# Autodesk Inventor assembly: suspensionsystem1
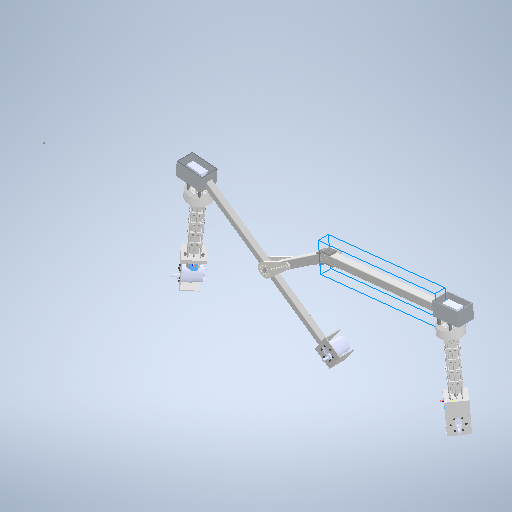
[picture p0: Inventor's stored thumbnail of the model, 512x512]
Saved by Autodesk Inventor 2025.4 (Build 294407000, 407)
## iProperties
Created: 2026-03-25
Part Number: suspensionsystem1
Document SubType Name: Assembly
Designer: hp
Author: hp
## Documents named in this file (51)
- C:\Users\hp\OneDrive\Desktop\Probitymechanicaldocs\suspensionsystem1.iam
- C:\Users\hp\OneDrive\Desktop\Probitymechanicaldocs\suspensionarms.ipt
- C:\Users\hp\OneDrive\Desktop\Probitymechanicaldocs\suspensionaxlebearing.ipt
- C:\Users\hp\OneDrive\Desktop\Probitymechanicaldocs\Controlarm.ipt
- C:\Users\hp\OneDrive\Desktop\Probitymechanicaldocs\rockershaft.ipt
- C:\Users\hp\OneDrive\Desktop\Probitymechanicaldocs\rockerwasher.ipt
- C:\Users\hp\OneDrive\Desktop\Probitymechanicaldocs\suspension2chassisarm.ipt
- C:\Users\hp\OneDrive\Desktop\Probitymechanicaldocs\150degreebracket.ipt
- C:\Users\hp\OneDrive\Desktop\Probitymechanicaldocs\rockerpivotarm.ipt
- C:\Users\hp\OneDrive\Desktop\Probitymechanicaldocs\finalturnmotorcasing.ipt
- C:\Users\hp\OneDrive\Desktop\Probitymechanicaldocs\finalturnmotorservo.ipt
- C:\Users\hp\OneDrive\Desktop\Probitymechanicaldocs\hexcoupling.ipt
- C:\Users\hp\OneDrive\Desktop\Probitymechanicaldocs\couplingload.ipt
- C:\Users\hp\OneDrive\Desktop\Probitymechanicaldocs\sleeve.ipt
- C:\Users\hp\OneDrive\Desktop\Probitymechanicaldocs\verticalaxle.ipt
- C:\Users\hp\OneDrive\Desktop\Probitymechanicaldocs\leadscrew.ipt
- C:\Users\hp\OneDrive\Desktop\Probitymechanicaldocs\leadscrewaxle.ipt
- C:\Users\hp\OneDrive\Desktop\Probitymechanicaldocs\RISE&Fallmotor.ipt
- C:\Users\hp\OneDrive\Desktop\Probitymechanicaldocs\spokes.ipt
- C:\Users\hp\OneDrive\Desktop\Probitymechanicaldocs\liftmotorfloor.ipt
- C:\Users\hp\OneDrive\Desktop\Probitymechanicaldocs\placeholderjoint.ipt
- C:\Users\hp\OneDrive\Desktop\Probitymechanicaldocs\impromptugraphitering.ipt
- C:\Users\hp\OneDrive\Desktop\Probitymechanicaldocs\Placeholderjointouterring.ipt
- C:\Users\hp\OneDrive\Desktop\Probitymechanicaldocs\drivemotorcasing.ipt
- C:\Users\hp\OneDrive\Desktop\Probitymechanicaldocs\extendeddrivemotorcasing.ipt
- C:\Users\hp\OneDrive\Desktop\Probitymechanicaldocs\finaldrivemotor.ipt
- C:\Users\hp\OneDrive\Desktop\Probitymechanicaldocs\150degreesidebracker.ipt
- C:\Users\hp\OneDrive\Documents\Inventor\Content Center Files\R2025\en-US\ISO 4762(2)\ISO 4762 - M4 x 6ISO.ipt
- C:\Users\hp\OneDrive\Documents\Inventor\Content Center Files\R2025\en-US\ISO 7045  H\ISO 7045 - M2.5 x 3_ - 4.8 - H - ISO.ipt
- C:\Users\hp\OneDrive\Documents\Inventor\Content Center Files\R2025\en-US\ISO 1580\ISO 1580 - M2 x 2.5_.ipt
- C:\Users\hp\OneDrive\Desktop\Probitymechanicaldocs\unusedparts\intermediatepin.ipt
- C:\Users\hp\OneDrive\Documents\Inventor\Content Center Files\R2025\en-US\ISO 4035(2)\ISO 4035 - M6 - ISO.ipt
- C:\Users\hp\OneDrive\Desktop\Probitymechanicaldocs\finalturnmotorcasing_MIR.ipt
- C:\Users\hp\OneDrive\Desktop\Probitymechanicaldocs\finalturnmotorservo_MIR.ipt
- C:\Users\hp\OneDrive\Desktop\Probitymechanicaldocs\hexcoupling_MIR.ipt
- C:\Users\hp\OneDrive\Desktop\Probitymechanicaldocs\couplingload_MIR.ipt
- C:\Users\hp\OneDrive\Desktop\Probitymechanicaldocs\sleeve_MIR.ipt
- C:\Users\hp\OneDrive\Desktop\Probitymechanicaldocs\verticalaxle_MIR.ipt
- C:\Users\hp\OneDrive\Desktop\Probitymechanicaldocs\leadscrew_MIR.ipt
- C:\Users\hp\OneDrive\Desktop\Probitymechanicaldocs\leadscrewaxle_MIR.ipt
- C:\Users\hp\OneDrive\Desktop\Probitymechanicaldocs\RISE&Fallmotor_MIR.ipt
- C:\Users\hp\OneDrive\Desktop\Probitymechanicaldocs\spokes_MIR.ipt
- C:\Users\hp\OneDrive\Desktop\Probitymechanicaldocs\liftmotorfloor_MIR.ipt
- C:\Users\hp\OneDrive\Desktop\Probitymechanicaldocs\placeholderjoint_MIR.ipt
- C:\Users\hp\OneDrive\Desktop\Probitymechanicaldocs\impromptugraphitering_MIR.ipt
- C:\Users\hp\OneDrive\Desktop\Probitymechanicaldocs\Placeholderjointouterring_MIR.ipt
- C:\Users\hp\OneDrive\Desktop\Probitymechanicaldocs\extendeddrivemotorcasing_MIR.ipt
- C:\Users\hp\OneDrive\Desktop\Probitymechanicaldocs\finaldrivemotor_MIR.ipt
- C:\Users\hp\OneDrive\Desktop\Probitymechanicaldocs\unusedparts\intermediatepin_MIR.ipt
- C:\Users\hp\OneDrive\Desktop\Probitymechanicaldocs\suspension2chassiscylindricalshaft.ipt
- C:\Users\hp\OneDrive\Desktop\Probitymechanicaldocs\suspension2chassiscylindricalpins.ipt
## Components (217 placed, 50 different names)
1. suspensionarms:1 — Rigid:8, Rotational:130, Rigid:41
2. suspensionaxlebearing:1 — Rotational:3
3. suspensionaxlebearing:2 — Cylindrical:1, Rotational:4, Rotational:130
4. Controlarm:1 — Rotational:9, Rotational:11, Rotational:131
5. Controlarm:2 — Cylindrical:11, Rotational:12, Rotational:132
6. rockershaft:1 — Cylindrical:1
7. rockerwasher:1 — Rotational:4, Rotational:6
8. rockerwasher:2 — Rotational:3, Rotational:5
9. suspensionaxlebearing:3 — Rotational:6, Rotational:11
10. suspensionaxlebearing:4 — Rotational:5, Cylindrical:11
11. suspension2chassisarm:1 — Rotational:9, Rotational:12, Rotational:72, Rotational:131, Rotational:132
12. 150degreebracket:1 — Rigid:16, Rotational:72, Rigid:33
13. rockerpivotarm:1 — Rigid:1, Rigid:16, Rotational:159
14. finalturnmotorcasing:1 — Rigid:1, Rigid:2, Mate:8, Insert:57, Mate:10, Mate:12, Mate:14, Mate:15, Mate:16, Mate:18, Mate:20
15. finalturnmotorservo:1 — Rigid:2, Rotational:13
16. hexcoupling:1 — Rotational:13, Rigid:3
17. couplingload:1 — Rigid:3, Rigid:4
18. sleeve:1 — Rotational:14, Rotational:15, Insert:113, Insert:114, Insert:123, Insert:124, Insert:133, Insert:134, Insert:151, Insert:152
19. verticalaxle:1 — Rigid:4, Rotational:14, Rotational:15, Rotational:16, Cylindrical:12, Rotational:17, Cylindrical:13, Rotational:18, Cylindrical:14, Rotational:19, Rigid:6, Rotational:29, Rotational:30, Rotational:31, Insert:153, Insert:154, Insert:155, Insert:156
20. leadscrew:1 — Rigid:6, Cylindrical:15
21. leadscrewaxle:1 — Rigid:5, Cylindrical:15
22. RISE&Fallmotor:1 — Rigid:5, Rotational:32, Rotational:33
23. sleeve:2 — Rotational:18, Cylindrical:14, Insert:119, Insert:120, Insert:129, Insert:130, Insert:139, Insert:140, Insert:145, Insert:146
24. sleeve:3 — Rotational:19, Rotational:29, Insert:115, Insert:116, Insert:125, Insert:126, Insert:135, Insert:136, Insert:149, Insert:150
25. sleeve:4 — Rotational:17, Cylindrical:13, Insert:121, Insert:122, Insert:131, Insert:132, Insert:141, Insert:142, Insert:143, Insert:144
26. sleeve:5 — Rotational:16, Cylindrical:12, Rigid:7
27. sleeve:6 — Rotational:30, Rotational:31, Insert:117, Insert:118, Insert:127, Insert:128, Insert:137, Insert:138, Insert:147, Insert:148
28. spokes:1 — Rotational:24
29. spokes:2 — Rotational:25
30. spokes:3 — Rotational:23
31. spokes:4 — Rotational:26
32. spokes:5 — Rotational:22
33. spokes:6 — Rotational:28
34. spokes:7 — Rotational:21
35. spokes:8 — Rotational:27
36. liftmotorfloor:1 — Rotational:21, Rotational:22, Rotational:23, Rotational:24, Rotational:25, Rotational:26, Rotational:27, Rotational:28, Rotational:32, Rotational:33, Rotational:62, Mate:5
37. placeholderjoint:1 — Rigid:7, Rotational:34
38. impromptugraphitering:1 — Rotational:34, Rotational:35, Rotational:102
39. Placeholderjointouterring:1 — Rotational:102, Insert:49, Insert:50, Insert:51, Insert:52
40. Placeholderjointouterring:2 — Rotational:35
41. drivemotorcasing:1 — Rigid:8, Rotational:63, Rotational:64, Insert:11, Insert:12, Insert:13, Insert:14, Insert:15, Insert:16
42. extendeddrivemotorcasing:1 — Rotational:62, Mate:5, Rotational:65, Rotational:66, Insert:17, Insert:18, Insert:19, Insert:20, Insert:21, Insert:22
43. finaldrivemotor:1 — Rotational:65, Rotational:66
44. finaldrivemotor:2 — Rotational:63, Rotational:64
45. 150degreesidebracker:1 — Rigid:33, Rigid:43
46. ISO 4762 M4 x 6:1
47. ISO 4762 M4 x 6:2
48. ISO 7045 H M2.5 x 3 - 4.8 - H:7 — Insert:11
49. ISO 7045 H M2.5 x 3 - 4.8 - H:8 — Insert:12
50. ISO 7045 H M2.5 x 3 - 4.8 - H:9 — Insert:13
51. ISO 7045 H M2.5 x 3 - 4.8 - H:10 — Insert:14
52. ISO 7045 H M2.5 x 3 - 4.8 - H:11 — Insert:15
53. ISO 7045 H M2.5 x 3 - 4.8 - H:12 — Insert:16
54. ISO 7045 H M2.5 x 3 - 4.8 - H:13 — Insert:17
55. ISO 7045 H M2.5 x 3 - 4.8 - H:14 — Insert:18
56. ISO 7045 H M2.5 x 3 - 4.8 - H:15 — Insert:19
57. ISO 7045 H M2.5 x 3 - 4.8 - H:16 — Insert:20
58. ISO 7045 H M2.5 x 3 - 4.8 - H:17 — Insert:21
59. ISO 7045 H M2.5 x 3 - 4.8 - H:18 — Insert:22
60. ISO 1580 M2 x 2.5:3
61. ISO 1580 M2 x 2.5:4
62. ISO 1580 M2 x 2.5:5
63. ISO 1580 M2 x 2.5:26
64. intermediatepin:1 — Insert:49, Mate:11, Mate:13
65. intermediatepin:2 — Insert:50, Mate:9
66. intermediatepin:3 — Insert:52, Mate:7, Mate:19
67. intermediatepin:5 — Insert:51, Mate:17
68. ISO 4035 M6:1 — Mate:7, Mate:8
69. ISO 4035 M6:2 — Insert:57
70. ISO 4035 M6:3 — Mate:9, Mate:10
71. ISO 4035 M6:4 — Mate:11, Mate:12
72. ISO 4035 M6:5 — Mate:13, Mate:14
73. ISO 4035 M6:6 — Mate:15, Mate:16
74. ISO 4035 M6:7 — Mate:17, Mate:18
75. ISO 4035 M6:8 — Mate:19, Mate:20
76. finalturnmotorcasing_MIR:1 — Mate:22, Insert:68, Mate:24, Mate:26, Mate:28, Mate:30, Mate:31, Mate:32, Mate:34, Rigid:35, Cylindrical:20, Cylindrical:21, Cylindrical:22, Rigid:41
77. finalturnmotorservo_MIR:1 — Rigid:35, Rotational:133
78. hexcoupling_MIR:1 — Rotational:133, Rigid:36
79. couplingload_MIR:1 — Rigid:36, Rigid:37
80. sleeve_MIR:1 — Rotational:134, Rotational:135, Insert:77, Insert:78, Insert:79, Insert:80, Insert:93, Insert:94, Insert:103, Insert:104
81. verticalaxle_MIR:1 — Rotational:134, Rotational:135, Rigid:37, Rigid:38, Cylindrical:17, Rotational:136, Rotational:137, Rotational:138, Cylindrical:18, Rotational:139, Cylindrical:19, Rotational:140, Rotational:141, Rotational:142, Insert:105, Insert:106, Insert:107, Insert:108
82. leadscrew_MIR:1 — Rigid:38, Cylindrical:16
83. leadscrewaxle_MIR:1 — Cylindrical:16, Rigid:39
84. RISE&Fallmotor_MIR:1 — Rigid:39, Rotational:143, Rotational:144
85. sleeve_MIR:2 — Cylindrical:17, Rotational:136, Insert:71, Insert:72, Insert:85, Insert:86, Insert:87, Insert:88, Insert:97, Insert:98
86. sleeve_MIR:3 — Rotational:137, Rotational:138, Insert:75, Insert:76, Insert:81, Insert:82, Insert:91, Insert:92, Insert:101, Insert:102
87. sleeve_MIR:4 — Cylindrical:18, Rotational:139, Insert:69, Insert:70, Insert:95, Insert:96, Insert:111, Insert:112
88. sleeve_MIR:5 — Cylindrical:19, Rotational:140, Rigid:40
89. sleeve_MIR:6 — Rotational:141, Rotational:142, Insert:73, Insert:74, Insert:83, Insert:84, Insert:89, Insert:90, Insert:99, Insert:100
90. spokes_MIR:1 — Rotational:149
91. spokes_MIR:2 — Rotational:148
92. spokes_MIR:3 — Rotational:150
93. spokes_MIR:4 — Rotational:147
94. spokes_MIR:5 — Rotational:151
95. spokes_MIR:6 — Rotational:145
96. spokes_MIR:7 — Rotational:152
97. spokes_MIR:8 — Rotational:146
98. liftmotorfloor_MIR:1 — Mate:21, Rotational:143, Rotational:144, Rotational:145, Rotational:146, Rotational:147, Rotational:148, Rotational:149, Rotational:150, Rotational:151, Rotational:152, Rotational:156, Insert:109, Insert:110
99. placeholderjoint_MIR:1 — Rigid:40, Rotational:153
100. impromptugraphitering_MIR:1 — Rotational:153, Rotational:154, Rotational:155
101. Placeholderjointouterring_MIR:1 — Insert:64, Insert:65, Insert:66, Insert:67, Rotational:154
102. Placeholderjointouterring_MIR:2 — Rotational:155
103. extendeddrivemotorcasing_MIR:1 — Mate:21, Insert:58, Insert:59, Insert:60, Insert:61, Insert:62, Insert:63, Rotational:156, Rotational:157, Rotational:158
104. finaldrivemotor_MIR:1 — Rotational:157, Rotational:158
105. ISO 7045 H M2.5 x 3 - 4.8 - H:19 — Insert:58
106. ISO 7045 H M2.5 x 3 - 4.8 - H:20 — Insert:59
107. ISO 7045 H M2.5 x 3 - 4.8 - H:21 — Insert:60
108. ISO 7045 H M2.5 x 3 - 4.8 - H:22 — Insert:61
109. ISO 7045 H M2.5 x 3 - 4.8 - H:23 — Insert:62
110. ISO 7045 H M2.5 x 3 - 4.8 - H:24 — Insert:63
111. intermediatepin_MIR:1 — Insert:64, Mate:27, Mate:29, Cylindrical:21
112. intermediatepin_MIR:2 — Insert:65, Mate:25, Cylindrical:20
113. intermediatepin_MIR:3 — Insert:66, Mate:23, Mate:35, Cylindrical:22
114. intermediatepin_MIR:4 — Insert:67, Mate:33
115. ISO 4035 M6:9 — Mate:22, Mate:23
116. ISO 4035 M6:10 — Insert:68
117. ISO 4035 M6:11 — Mate:24, Mate:25
118. ISO 4035 M6:12 — Mate:26, Mate:27
119. ISO 4035 M6:13 — Mate:28, Mate:29
120. ISO 4035 M6:14 — Mate:30, Mate:31
121. ISO 4035 M6:15 — Mate:32, Mate:33
122. ISO 4035 M6:16 — Mate:34, Mate:35
123. ISO 1580 M2 x 2.5:73
124. ISO 1580 M2 x 2.5:95 — Insert:69
125. ISO 1580 M2 x 2.5:96 — Insert:70
126. ISO 1580 M2 x 2.5:97 — Insert:71
127. ISO 1580 M2 x 2.5:98 — Insert:72
128. ISO 1580 M2 x 2.5:99 — Insert:73
129. ISO 1580 M2 x 2.5:100 — Insert:74
130. ISO 1580 M2 x 2.5:101 — Insert:75
131. ISO 1580 M2 x 2.5:102 — Insert:76
132. ISO 1580 M2 x 2.5:103 — Insert:77
133. ISO 1580 M2 x 2.5:104 — Insert:78
134. ISO 1580 M2 x 2.5:105 — Insert:79
135. ISO 1580 M2 x 2.5:106 — Insert:80
136. ISO 1580 M2 x 2.5:107 — Insert:81
137. ISO 1580 M2 x 2.5:108 — Insert:82
138. ISO 1580 M2 x 2.5:109 — Insert:83
139. ISO 1580 M2 x 2.5:110 — Insert:84
140. ISO 1580 M2 x 2.5:111 — Insert:85
141. ISO 1580 M2 x 2.5:112 — Insert:86
142. ISO 1580 M2 x 2.5:113 — Insert:87
143. ISO 1580 M2 x 2.5:114 — Insert:88
144. ISO 1580 M2 x 2.5:115 — Insert:89
145. ISO 1580 M2 x 2.5:116 — Insert:90
146. ISO 1580 M2 x 2.5:117 — Insert:91
147. ISO 1580 M2 x 2.5:118 — Insert:92
148. ISO 1580 M2 x 2.5:119 — Insert:93
149. ISO 1580 M2 x 2.5:120 — Insert:94
150. ISO 1580 M2 x 2.5:121 — Insert:95
151. ISO 1580 M2 x 2.5:122 — Insert:96
152. ISO 1580 M2 x 2.5:123 — Insert:97
153. ISO 1580 M2 x 2.5:124 — Insert:98
154. ISO 1580 M2 x 2.5:125 — Insert:99
155. ISO 1580 M2 x 2.5:126 — Insert:100
156. ISO 1580 M2 x 2.5:127 — Insert:101
157. ISO 1580 M2 x 2.5:128 — Insert:102
158. ISO 1580 M2 x 2.5:129 — Insert:103
159. ISO 1580 M2 x 2.5:130 — Insert:104
160. ISO 1580 M2 x 2.5:131 — Insert:105
161. ISO 1580 M2 x 2.5:132 — Insert:106
162. ISO 1580 M2 x 2.5:133 — Insert:107
163. ISO 1580 M2 x 2.5:134 — Insert:108
164. ISO 4762 M4 x 6:5 — Insert:109
165. ISO 4762 M4 x 6:6 — Insert:110
166. suspension2chassiscylindricalshaft:1 — Rotational:159, Rotational:160, Rotational:161, Rotational:162, Rigid:42
167. suspension2chassiscylindricalpins:1 — Rotational:162
168. suspension2chassiscylindricalpins:2 — Rotational:160
169. suspension2chassiscylindricalpins:3 — Rotational:161
170. suspension2chassiscylindricalpins:4 — Rigid:42
171. 150degreebracket:2 — Rigid:43
172. ISO 1580 M2 x 2.5:135 — Insert:111
173. ISO 1580 M2 x 2.5:136 — Insert:112
174. ISO 1580 M2 x 2.5:137 — Insert:113
175. ISO 1580 M2 x 2.5:138 — Insert:114
176. ISO 1580 M2 x 2.5:139 — Insert:115
177. ISO 1580 M2 x 2.5:140 — Insert:116
178. ISO 1580 M2 x 2.5:141 — Insert:117
179. ISO 1580 M2 x 2.5:142 — Insert:118
180. ISO 1580 M2 x 2.5:143 — Insert:119
181. ISO 1580 M2 x 2.5:144 — Insert:120
182. ISO 1580 M2 x 2.5:145 — Insert:121
183. ISO 1580 M2 x 2.5:146 — Insert:122
184. ISO 1580 M2 x 2.5:147 — Insert:123
185. ISO 1580 M2 x 2.5:148 — Insert:124
186. ISO 1580 M2 x 2.5:149 — Insert:125
187. ISO 1580 M2 x 2.5:150 — Insert:126
188. ISO 1580 M2 x 2.5:151 — Insert:127
189. ISO 1580 M2 x 2.5:152 — Insert:128
190. ISO 1580 M2 x 2.5:153 — Insert:129
191. ISO 1580 M2 x 2.5:154 — Insert:130
192. ISO 1580 M2 x 2.5:155 — Insert:131
193. ISO 1580 M2 x 2.5:156 — Insert:132
194. ISO 1580 M2 x 2.5:157 — Insert:133
195. ISO 1580 M2 x 2.5:158 — Insert:134
196. ISO 1580 M2 x 2.5:159 — Insert:135
197. ISO 1580 M2 x 2.5:160 — Insert:136
198. ISO 1580 M2 x 2.5:161 — Insert:137
199. ISO 1580 M2 x 2.5:162 — Insert:138
200. ISO 1580 M2 x 2.5:163 — Insert:139
201. ISO 1580 M2 x 2.5:164 — Insert:140
202. ISO 1580 M2 x 2.5:165 — Insert:141
203. ISO 1580 M2 x 2.5:166 — Insert:142
204. ISO 1580 M2 x 2.5:167 — Insert:143
205. ISO 1580 M2 x 2.5:168 — Insert:144
206. ISO 1580 M2 x 2.5:169 — Insert:145
207. ISO 1580 M2 x 2.5:170 — Insert:146
208. ISO 1580 M2 x 2.5:171 — Insert:147
209. ISO 1580 M2 x 2.5:172 — Insert:148
210. ISO 1580 M2 x 2.5:173 — Insert:149
211. ISO 1580 M2 x 2.5:174 — Insert:150
212. ISO 1580 M2 x 2.5:175 — Insert:151
213. ISO 1580 M2 x 2.5:176 — Insert:152
214. ISO 1580 M2 x 2.5:177 — Insert:153
215. ISO 1580 M2 x 2.5:178 — Insert:154
216. ISO 1580 M2 x 2.5:179 — Insert:155
217. ISO 1580 M2 x 2.5:180 — Insert:156
## Relationships (247: Insert 116, RevoluteJoint 69, Mate 30, WeldJoint 19, CylindricalJoint 13)
- Cylindrical:1: suspensionaxlebearing:2 ↔ rockershaft:1
- Rotational:3 [RevoluteJoint]: suspensionaxlebearing:1 ↔ rockerwasher:2
- Rotational:4 [RevoluteJoint]: suspensionaxlebearing:2 ↔ rockerwasher:1
- Rotational:5 [RevoluteJoint]: rockerwasher:2 ↔ suspensionaxlebearing:4
- Rotational:6 [RevoluteJoint]: rockerwasher:1 ↔ suspensionaxlebearing:3
- Rotational:9 [RevoluteJoint]: Controlarm:1 ↔ suspension2chassisarm:1
- Cylindrical:11: Controlarm:2 ↔ suspensionaxlebearing:4
- Rotational:11 [RevoluteJoint]: Controlarm:1 ↔ suspensionaxlebearing:3
- Rotational:12 [RevoluteJoint]: Controlarm:2 ↔ suspension2chassisarm:1
- Rigid:1 [WeldJoint]: rockerpivotarm:1 ↔ finalturnmotorcasing:1
- Rigid:2 [WeldJoint]: finalturnmotorcasing:1 ↔ finalturnmotorservo:1
- Rotational:13 [RevoluteJoint]: finalturnmotorservo:1 ↔ hexcoupling:1
- Rigid:3 [WeldJoint]: hexcoupling:1 ↔ couplingload:1
- Rigid:4 [WeldJoint]: couplingload:1 ↔ verticalaxle:1
- Rotational:14 [RevoluteJoint]: sleeve:1 ↔ verticalaxle:1
- Rotational:15 [RevoluteJoint]: sleeve:1 ↔ verticalaxle:1
- Rotational:16 [RevoluteJoint]: verticalaxle:1 ↔ sleeve:5
- Cylindrical:12: verticalaxle:1 ↔ sleeve:5
- Rotational:17 [RevoluteJoint]: verticalaxle:1 ↔ sleeve:4
- Cylindrical:13: verticalaxle:1 ↔ sleeve:4
- Rotational:18 [RevoluteJoint]: verticalaxle:1 ↔ sleeve:2
- Cylindrical:14: verticalaxle:1 ↔ sleeve:2
- Rotational:19 [RevoluteJoint]: verticalaxle:1 ↔ sleeve:3
- Rigid:5 [WeldJoint] (-4 mm): leadscrewaxle:1 ↔ RISE&Fallmotor:1
- Rigid:6 [WeldJoint]: verticalaxle:1 ↔ leadscrew:1
- Cylindrical:15: leadscrew:1 ↔ leadscrewaxle:1
- Rotational:21 [RevoluteJoint] (8 mm): spokes:7 ↔ liftmotorfloor:1
- Rotational:22 [RevoluteJoint] (8 mm): spokes:5 ↔ liftmotorfloor:1
- Rotational:23 [RevoluteJoint] (8 mm): spokes:3 ↔ liftmotorfloor:1
- Rotational:24 [RevoluteJoint] (8 mm): spokes:1 ↔ liftmotorfloor:1
- Rotational:25 [RevoluteJoint] (8 mm): spokes:2 ↔ liftmotorfloor:1
- Rotational:26 [RevoluteJoint] (8 mm): spokes:4 ↔ liftmotorfloor:1
- Rotational:27 [RevoluteJoint] (8 mm): spokes:8 ↔ liftmotorfloor:1
- Rotational:28 [RevoluteJoint] (8 mm): spokes:6 ↔ liftmotorfloor:1
- Rotational:29 [RevoluteJoint]: verticalaxle:1 ↔ sleeve:3
- Rotational:30 [RevoluteJoint]: verticalaxle:1 ↔ sleeve:6
- Rotational:31 [RevoluteJoint]: verticalaxle:1 ↔ sleeve:6
- Rotational:32 [RevoluteJoint]: RISE&Fallmotor:1 ↔ liftmotorfloor:1
- Rotational:33 [RevoluteJoint]: RISE&Fallmotor:1 ↔ liftmotorfloor:1
- Rigid:7 [WeldJoint]: sleeve:5 ↔ placeholderjoint:1
- Rotational:34 [RevoluteJoint]: placeholderjoint:1 ↔ impromptugraphitering:1
- Rotational:35 [RevoluteJoint]: impromptugraphitering:1 ↔ Placeholderjointouterring:2
- Rigid:8 [WeldJoint]: suspensionarms:1 ↔ drivemotorcasing:1
- Rotational:62 [RevoluteJoint]: liftmotorfloor:1 ↔ extendeddrivemotorcasing:1
- Mate:5: liftmotorfloor:1 ↔ extendeddrivemotorcasing:1
- Rotational:63 [RevoluteJoint]: drivemotorcasing:1 ↔ finaldrivemotor:2
- Rotational:64 [RevoluteJoint]: drivemotorcasing:1 ↔ finaldrivemotor:2
- Rotational:65 [RevoluteJoint]: extendeddrivemotorcasing:1 ↔ finaldrivemotor:1
- Rotational:66 [RevoluteJoint]: extendeddrivemotorcasing:1 ↔ finaldrivemotor:1
- Rigid:16 [WeldJoint]: 150degreebracket:1 ↔ rockerpivotarm:1
- Rotational:72 [RevoluteJoint]: suspension2chassisarm:1 ↔ 150degreebracket:1
- Rotational:102 [RevoluteJoint]: impromptugraphitering:1 ↔ Placeholderjointouterring:1
- Rotational:130 [RevoluteJoint]: suspensionarms:1 ↔ suspensionaxlebearing:2
- Rotational:131 [RevoluteJoint]: Controlarm:1 ↔ suspension2chassisarm:1
- Rotational:132 [RevoluteJoint]: Controlarm:2 ↔ suspension2chassisarm:1
- Insert:11: drivemotorcasing:1 ↔ ISO 7045 H M2.5 x 3 - 4.8 - H:7
- Insert:12: drivemotorcasing:1 ↔ ISO 7045 H M2.5 x 3 - 4.8 - H:8
- Insert:13: drivemotorcasing:1 ↔ ISO 7045 H M2.5 x 3 - 4.8 - H:9
- Insert:14: drivemotorcasing:1 ↔ ISO 7045 H M2.5 x 3 - 4.8 - H:10
- Insert:15: drivemotorcasing:1 ↔ ISO 7045 H M2.5 x 3 - 4.8 - H:11
- Insert:16: drivemotorcasing:1 ↔ ISO 7045 H M2.5 x 3 - 4.8 - H:12
- Insert:17: extendeddrivemotorcasing:1 ↔ ISO 7045 H M2.5 x 3 - 4.8 - H:13
- Insert:18: extendeddrivemotorcasing:1 ↔ ISO 7045 H M2.5 x 3 - 4.8 - H:14
- Insert:19: extendeddrivemotorcasing:1 ↔ ISO 7045 H M2.5 x 3 - 4.8 - H:15
- Insert:20: extendeddrivemotorcasing:1 ↔ ISO 7045 H M2.5 x 3 - 4.8 - H:16
- Insert:21: extendeddrivemotorcasing:1 ↔ ISO 7045 H M2.5 x 3 - 4.8 - H:17
- Insert:22: extendeddrivemotorcasing:1 ↔ ISO 7045 H M2.5 x 3 - 4.8 - H:18
- Rigid:33 [WeldJoint]: 150degreebracket:1 ↔ 150degreesidebracker:1
- Insert:49 (-5 mm): Placeholderjointouterring:1 ↔ intermediatepin:1
- Insert:50 (-5 mm): Placeholderjointouterring:1 ↔ intermediatepin:2
- Insert:51 (-5 mm): Placeholderjointouterring:1 ↔ intermediatepin:5
- Insert:52 (-5 mm): Placeholderjointouterring:1 ↔ intermediatepin:3
- Mate:7: intermediatepin:3 ↔ ISO 4035 M6:1
- Mate:8: finalturnmotorcasing:1 ↔ ISO 4035 M6:1
- Insert:57: finalturnmotorcasing:1 ↔ ISO 4035 M6:2
- Mate:9: intermediatepin:2 ↔ ISO 4035 M6:3
- Mate:10: finalturnmotorcasing:1 ↔ ISO 4035 M6:3
- Mate:11: intermediatepin:1 ↔ ISO 4035 M6:4
- Mate:12: finalturnmotorcasing:1 ↔ ISO 4035 M6:4
- Mate:13: intermediatepin:1 ↔ ISO 4035 M6:5
- Mate:14: finalturnmotorcasing:1 ↔ ISO 4035 M6:5
- Mate:15: finalturnmotorcasing:1 ↔ ISO 4035 M6:6
- Mate:16: finalturnmotorcasing:1 ↔ ISO 4035 M6:6
- Mate:17: intermediatepin:5 ↔ ISO 4035 M6:7
- Mate:18: finalturnmotorcasing:1 ↔ ISO 4035 M6:7
- Mate:19: intermediatepin:3 ↔ ISO 4035 M6:8
- Mate:20: finalturnmotorcasing:1 ↔ ISO 4035 M6:8
- Mate:21: liftmotorfloor_MIR:1 ↔ extendeddrivemotorcasing_MIR:1
- Insert:58: extendeddrivemotorcasing_MIR:1 ↔ ISO 7045 H M2.5 x 3 - 4.8 - H:19
- Insert:59: extendeddrivemotorcasing_MIR:1 ↔ ISO 7045 H M2.5 x 3 - 4.8 - H:20
- Insert:60: extendeddrivemotorcasing_MIR:1 ↔ ISO 7045 H M2.5 x 3 - 4.8 - H:21
- Insert:61: extendeddrivemotorcasing_MIR:1 ↔ ISO 7045 H M2.5 x 3 - 4.8 - H:22
- Insert:62: extendeddrivemotorcasing_MIR:1 ↔ ISO 7045 H M2.5 x 3 - 4.8 - H:23
- Insert:63: extendeddrivemotorcasing_MIR:1 ↔ ISO 7045 H M2.5 x 3 - 4.8 - H:24
- Insert:64 (-5 mm): Placeholderjointouterring_MIR:1 ↔ intermediatepin_MIR:1
- Insert:65 (-5 mm): Placeholderjointouterring_MIR:1 ↔ intermediatepin_MIR:2
- Insert:66 (-5 mm): Placeholderjointouterring_MIR:1 ↔ intermediatepin_MIR:3
- Insert:67 (-5 mm): Placeholderjointouterring_MIR:1 ↔ intermediatepin_MIR:4
- Mate:22: finalturnmotorcasing_MIR:1 ↔ ISO 4035 M6:9
- Mate:23: intermediatepin_MIR:3 ↔ ISO 4035 M6:9
- Insert:68: finalturnmotorcasing_MIR:1 ↔ ISO 4035 M6:10
- Mate:24: finalturnmotorcasing_MIR:1 ↔ ISO 4035 M6:11
- Mate:25: intermediatepin_MIR:2 ↔ ISO 4035 M6:11
- Mate:26: finalturnmotorcasing_MIR:1 ↔ ISO 4035 M6:12
- Mate:27: intermediatepin_MIR:1 ↔ ISO 4035 M6:12
- Mate:28: finalturnmotorcasing_MIR:1 ↔ ISO 4035 M6:13
- Mate:29: intermediatepin_MIR:1 ↔ ISO 4035 M6:13
- Mate:30: finalturnmotorcasing_MIR:1 ↔ ISO 4035 M6:14
- Mate:31: finalturnmotorcasing_MIR:1 ↔ ISO 4035 M6:14
- Mate:32: finalturnmotorcasing_MIR:1 ↔ ISO 4035 M6:15
- Mate:33: intermediatepin_MIR:4 ↔ ISO 4035 M6:15
- Mate:34: finalturnmotorcasing_MIR:1 ↔ ISO 4035 M6:16
- Mate:35: intermediatepin_MIR:3 ↔ ISO 4035 M6:16
- Rigid:35 [WeldJoint]: finalturnmotorcasing_MIR:1 ↔ finalturnmotorservo_MIR:1
- Rotational:133 [RevoluteJoint]: finalturnmotorservo_MIR:1 ↔ hexcoupling_MIR:1
- Rigid:36 [WeldJoint]: hexcoupling_MIR:1 ↔ couplingload_MIR:1
- Rotational:134 [RevoluteJoint]: sleeve_MIR:1 ↔ verticalaxle_MIR:1
- Rotational:135 [RevoluteJoint]: sleeve_MIR:1 ↔ verticalaxle_MIR:1
- Rigid:37 [WeldJoint]: couplingload_MIR:1 ↔ verticalaxle_MIR:1
- Rigid:38 [WeldJoint]: verticalaxle_MIR:1 ↔ leadscrew_MIR:1
- Cylindrical:16: leadscrew_MIR:1 ↔ leadscrewaxle_MIR:1
- Rigid:39 [WeldJoint] (-4 mm): leadscrewaxle_MIR:1 ↔ RISE&Fallmotor_MIR:1
- Cylindrical:17: verticalaxle_MIR:1 ↔ sleeve_MIR:2
- Rotational:136 [RevoluteJoint]: verticalaxle_MIR:1 ↔ sleeve_MIR:2
- Rotational:137 [RevoluteJoint]: verticalaxle_MIR:1 ↔ sleeve_MIR:3
- Rotational:138 [RevoluteJoint]: verticalaxle_MIR:1 ↔ sleeve_MIR:3
- Cylindrical:18: verticalaxle_MIR:1 ↔ sleeve_MIR:4
- Rotational:139 [RevoluteJoint]: verticalaxle_MIR:1 ↔ sleeve_MIR:4
- Cylindrical:19: verticalaxle_MIR:1 ↔ sleeve_MIR:5
- Rotational:140 [RevoluteJoint]: verticalaxle_MIR:1 ↔ sleeve_MIR:5
- Rotational:141 [RevoluteJoint]: verticalaxle_MIR:1 ↔ sleeve_MIR:6
- Rotational:142 [RevoluteJoint]: verticalaxle_MIR:1 ↔ sleeve_MIR:6
- Rotational:143 [RevoluteJoint]: RISE&Fallmotor_MIR:1 ↔ liftmotorfloor_MIR:1
- Rotational:144 [RevoluteJoint]: RISE&Fallmotor_MIR:1 ↔ liftmotorfloor_MIR:1
- Rotational:145 [RevoluteJoint] (-8 mm): spokes_MIR:6 ↔ liftmotorfloor_MIR:1
- Rotational:146 [RevoluteJoint] (-8 mm): spokes_MIR:8 ↔ liftmotorfloor_MIR:1
- Rotational:147 [RevoluteJoint] (-8 mm): spokes_MIR:4 ↔ liftmotorfloor_MIR:1
- Rotational:148 [RevoluteJoint] (-8 mm): spokes_MIR:2 ↔ liftmotorfloor_MIR:1
- Rotational:149 [RevoluteJoint] (-8 mm): spokes_MIR:1 ↔ liftmotorfloor_MIR:1
- Rotational:150 [RevoluteJoint] (-8 mm): spokes_MIR:3 ↔ liftmotorfloor_MIR:1
- Rotational:151 [RevoluteJoint] (-8 mm): spokes_MIR:5 ↔ liftmotorfloor_MIR:1
- Rotational:152 [RevoluteJoint] (-8 mm): spokes_MIR:7 ↔ liftmotorfloor_MIR:1
- Rigid:40 [WeldJoint]: sleeve_MIR:5 ↔ placeholderjoint_MIR:1
- Rotational:153 [RevoluteJoint]: placeholderjoint_MIR:1 ↔ impromptugraphitering_MIR:1
- Rotational:154 [RevoluteJoint]: impromptugraphitering_MIR:1 ↔ Placeholderjointouterring_MIR:1
- Rotational:155 [RevoluteJoint]: impromptugraphitering_MIR:1 ↔ Placeholderjointouterring_MIR:2
- Rotational:156 [RevoluteJoint]: liftmotorfloor_MIR:1 ↔ extendeddrivemotorcasing_MIR:1
- Rotational:157 [RevoluteJoint]: extendeddrivemotorcasing_MIR:1 ↔ finaldrivemotor_MIR:1
- Rotational:158 [RevoluteJoint]: extendeddrivemotorcasing_MIR:1 ↔ finaldrivemotor_MIR:1
- Cylindrical:20: finalturnmotorcasing_MIR:1 ↔ intermediatepin_MIR:2
- Cylindrical:21: finalturnmotorcasing_MIR:1 ↔ intermediatepin_MIR:1
- Cylindrical:22: finalturnmotorcasing_MIR:1 ↔ intermediatepin_MIR:3
- Rigid:41 [WeldJoint]: suspensionarms:1 ↔ finalturnmotorcasing_MIR:1
- Insert:69: sleeve_MIR:4 ↔ ISO 1580 M2 x 2.5:95
- Insert:70: sleeve_MIR:4 ↔ ISO 1580 M2 x 2.5:96
- Insert:71: sleeve_MIR:2 ↔ ISO 1580 M2 x 2.5:97
- Insert:72: sleeve_MIR:2 ↔ ISO 1580 M2 x 2.5:98
- Insert:73: sleeve_MIR:6 ↔ ISO 1580 M2 x 2.5:99
- Insert:74: sleeve_MIR:6 ↔ ISO 1580 M2 x 2.5:100
- Insert:75: sleeve_MIR:3 ↔ ISO 1580 M2 x 2.5:101
- Insert:76: sleeve_MIR:3 ↔ ISO 1580 M2 x 2.5:102
- Insert:77: sleeve_MIR:1 ↔ ISO 1580 M2 x 2.5:103
- Insert:78: sleeve_MIR:1 ↔ ISO 1580 M2 x 2.5:104
- Insert:79: sleeve_MIR:1 ↔ ISO 1580 M2 x 2.5:105
- Insert:80: sleeve_MIR:1 ↔ ISO 1580 M2 x 2.5:106
- Insert:81: sleeve_MIR:3 ↔ ISO 1580 M2 x 2.5:107
- Insert:82: sleeve_MIR:3 ↔ ISO 1580 M2 x 2.5:108
- Insert:83: sleeve_MIR:6 ↔ ISO 1580 M2 x 2.5:109
- Insert:84: sleeve_MIR:6 ↔ ISO 1580 M2 x 2.5:110
- Insert:85: sleeve_MIR:2 ↔ ISO 1580 M2 x 2.5:111
- Insert:86: sleeve_MIR:2 ↔ ISO 1580 M2 x 2.5:112
- Insert:87: sleeve_MIR:2 ↔ ISO 1580 M2 x 2.5:113
- Insert:88: sleeve_MIR:2 ↔ ISO 1580 M2 x 2.5:114
- Insert:89: sleeve_MIR:6 ↔ ISO 1580 M2 x 2.5:115
- Insert:90: sleeve_MIR:6 ↔ ISO 1580 M2 x 2.5:116
- Insert:91: sleeve_MIR:3 ↔ ISO 1580 M2 x 2.5:117
- Insert:92: sleeve_MIR:3 ↔ ISO 1580 M2 x 2.5:118
- Insert:93: sleeve_MIR:1 ↔ ISO 1580 M2 x 2.5:119
- Insert:94: sleeve_MIR:1 ↔ ISO 1580 M2 x 2.5:120
- Insert:95: sleeve_MIR:4 ↔ ISO 1580 M2 x 2.5:121
- Insert:96: sleeve_MIR:4 ↔ ISO 1580 M2 x 2.5:122
- Insert:97: sleeve_MIR:2 ↔ ISO 1580 M2 x 2.5:123
- Insert:98: sleeve_MIR:2 ↔ ISO 1580 M2 x 2.5:124
- Insert:99: sleeve_MIR:6 ↔ ISO 1580 M2 x 2.5:125
- Insert:100: sleeve_MIR:6 ↔ ISO 1580 M2 x 2.5:126
- Insert:101: sleeve_MIR:3 ↔ ISO 1580 M2 x 2.5:127
- Insert:102: sleeve_MIR:3 ↔ ISO 1580 M2 x 2.5:128
- Insert:103: sleeve_MIR:1 ↔ ISO 1580 M2 x 2.5:129
- Insert:104: sleeve_MIR:1 ↔ ISO 1580 M2 x 2.5:130
- Insert:105: verticalaxle_MIR:1 ↔ ISO 1580 M2 x 2.5:131
- Insert:106: verticalaxle_MIR:1 ↔ ISO 1580 M2 x 2.5:132
- Insert:107: verticalaxle_MIR:1 ↔ ISO 1580 M2 x 2.5:133
- Insert:108: verticalaxle_MIR:1 ↔ ISO 1580 M2 x 2.5:134
- Insert:109: liftmotorfloor_MIR:1 ↔ ISO 4762 M4 x 6:5
- Insert:110: liftmotorfloor_MIR:1 ↔ ISO 4762 M4 x 6:6
- Rotational:159 [RevoluteJoint]: rockerpivotarm:1 ↔ suspension2chassiscylindricalshaft:1
- Rotational:160 [RevoluteJoint]: suspension2chassiscylindricalshaft:1 ↔ suspension2chassiscylindricalpins:2
- Rotational:161 [RevoluteJoint]: suspension2chassiscylindricalshaft:1 ↔ suspension2chassiscylindricalpins:3
- Rotational:162 [RevoluteJoint]: suspension2chassiscylindricalshaft:1 ↔ suspension2chassiscylindricalpins:1
- Rigid:42 [WeldJoint]: suspension2chassiscylindricalshaft:1 ↔ suspension2chassiscylindricalpins:4
- Rigid:43 [WeldJoint]: 150degreesidebracker:1 ↔ 150degreebracket:2
- Insert:111: sleeve_MIR:4 ↔ ISO 1580 M2 x 2.5:135
- Insert:112: sleeve_MIR:4 ↔ ISO 1580 M2 x 2.5:136
- Insert:113: sleeve:1 ↔ ISO 1580 M2 x 2.5:137
- Insert:114: sleeve:1 ↔ ISO 1580 M2 x 2.5:138
- Insert:115: sleeve:3 ↔ ISO 1580 M2 x 2.5:139
- Insert:116: sleeve:3 ↔ ISO 1580 M2 x 2.5:140
- Insert:117: sleeve:6 ↔ ISO 1580 M2 x 2.5:141
- Insert:118: sleeve:6 ↔ ISO 1580 M2 x 2.5:142
- Insert:119: sleeve:2 ↔ ISO 1580 M2 x 2.5:143
- Insert:120: sleeve:2 ↔ ISO 1580 M2 x 2.5:144
- Insert:121: sleeve:4 ↔ ISO 1580 M2 x 2.5:145
- Insert:122: sleeve:4 ↔ ISO 1580 M2 x 2.5:146
- Insert:123: sleeve:1 ↔ ISO 1580 M2 x 2.5:147
- Insert:124: sleeve:1 ↔ ISO 1580 M2 x 2.5:148
- Insert:125: sleeve:3 ↔ ISO 1580 M2 x 2.5:149
- Insert:126: sleeve:3 ↔ ISO 1580 M2 x 2.5:150
- Insert:127: sleeve:6 ↔ ISO 1580 M2 x 2.5:151
- Insert:128: sleeve:6 ↔ ISO 1580 M2 x 2.5:152
- Insert:129: sleeve:2 ↔ ISO 1580 M2 x 2.5:153
- Insert:130: sleeve:2 ↔ ISO 1580 M2 x 2.5:154
- Insert:131: sleeve:4 ↔ ISO 1580 M2 x 2.5:155
- Insert:132: sleeve:4 ↔ ISO 1580 M2 x 2.5:156
- Insert:133: sleeve:1 ↔ ISO 1580 M2 x 2.5:157
- Insert:134: sleeve:1 ↔ ISO 1580 M2 x 2.5:158
- Insert:135: sleeve:3 ↔ ISO 1580 M2 x 2.5:159
- Insert:136: sleeve:3 ↔ ISO 1580 M2 x 2.5:160
- Insert:137: sleeve:6 ↔ ISO 1580 M2 x 2.5:161
- Insert:138: sleeve:6 ↔ ISO 1580 M2 x 2.5:162
- Insert:139: sleeve:2 ↔ ISO 1580 M2 x 2.5:163
- Insert:140: sleeve:2 ↔ ISO 1580 M2 x 2.5:164
- Insert:141: sleeve:4 ↔ ISO 1580 M2 x 2.5:165
- Insert:142: sleeve:4 ↔ ISO 1580 M2 x 2.5:166
- Insert:143: sleeve:4 ↔ ISO 1580 M2 x 2.5:167
- Insert:144: sleeve:4 ↔ ISO 1580 M2 x 2.5:168
- Insert:145: sleeve:2 ↔ ISO 1580 M2 x 2.5:169
- Insert:146: sleeve:2 ↔ ISO 1580 M2 x 2.5:170
- Insert:147: sleeve:6 ↔ ISO 1580 M2 x 2.5:171
- Insert:148: sleeve:6 ↔ ISO 1580 M2 x 2.5:172
- Insert:149: sleeve:3 ↔ ISO 1580 M2 x 2.5:173
- Insert:150: sleeve:3 ↔ ISO 1580 M2 x 2.5:174
- Insert:151: sleeve:1 ↔ ISO 1580 M2 x 2.5:175
- Insert:152: sleeve:1 ↔ ISO 1580 M2 x 2.5:176
- Insert:153: verticalaxle:1 ↔ ISO 1580 M2 x 2.5:177
- Insert:154: verticalaxle:1 ↔ ISO 1580 M2 x 2.5:178
- Insert:155: verticalaxle:1 ↔ ISO 1580 M2 x 2.5:179
- Insert:156: verticalaxle:1 ↔ ISO 1580 M2 x 2.5:180
